# Autodesk Inventor assembly: Box_assembly
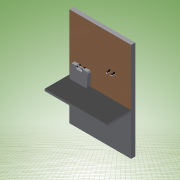
[picture p0: Inventor's stored thumbnail of the model, 180x180]
Saved by Autodesk Inventor 2017 (Build 210142000, 142)
## iProperties
Created: 2018-06-04
Part Number: Box_assembly
Document SubType Name: Assembly
Designer: Spark Electronics
Author: Spark Electronics
## Documents named in this file (5)
- C:\Users\Owner\Documents\SPARK RESEARCH\Projects\Organization\Divider Boxes\Box_assembly.iam
- C:\Users\Owner\Documents\SPARK RESEARCH\Projects\Organization\Divider Boxes\Wall_desk.ipt
- C:\Users\Owner\Documents\SPARK RESEARCH\Projects\Organization\Divider Boxes\Divider_box.ipt
- C:\Users\Owner\Documents\SPARK RESEARCH\Projects\Organization\Divider Boxes\wall_hook.ipt
- C:\Users\Owner\Documents\SPARK RESEARCH\Projects\Organization\Divider Boxes\Wall_mount.ipt
## Components (8 placed, 4 different names)
1. Wall_desk:1 — Mate:1, Mate:2, Flush:6, Mate:11, Mate:12
2. Divider_box:1 — Mate:5, Mate:7, Mate:8, Mate:9, Mate:10
3. wall_hook:1 — Flush:5, Mate:6, Mate:7, Mate:8, Mate:13, Mate:14, Mate:15
4. wall_hook:2 — Flush:5, Mate:5, Mate:6, Flush:6, Mate:9, Mate:10
5. wall_hook:3 — Mate:2
6. wall_hook:4 — Mate:1
7. Wall_mount:1 — Mate:12, Flush:7, Mate:13, Mate:14, Mate:15
8. Wall_mount:2 — Mate:11, Flush:7
## Relationships (16: Mate 13, Flush 3)
- Mate:1: Wall_desk:1 ↔ wall_hook:4
- Mate:2: Wall_desk:1 ↔ wall_hook:3
- Flush:5: wall_hook:1 ↔ wall_hook:2
- Mate:5: Divider_box:1 ↔ wall_hook:2
- Mate:6 (101.6 mm): wall_hook:1 ↔ wall_hook:2
- Mate:7 (0.254 mm): Divider_box:1 ↔ wall_hook:1
- Mate:8: Divider_box:1 ↔ wall_hook:1
- Flush:6 (381 mm): Wall_desk:1 ↔ wall_hook:2
- Mate:9 (6.35 mm): Divider_box:1 ↔ wall_hook:2
- Mate:10 (0.254 mm): Divider_box:1 ↔ wall_hook:2
- Mate:11: Wall_desk:1 ↔ Wall_mount:2
- Mate:12: Wall_desk:1 ↔ Wall_mount:1
- Flush:7 (6.35 mm): Wall_mount:1 ↔ Wall_mount:2
- Mate:13 (0.1 mm): wall_hook:1 ↔ Wall_mount:1
- Mate:14 (0.1 mm): wall_hook:1 ↔ Wall_mount:1
- Mate:15 (0.1 mm): wall_hook:1 ↔ Wall_mount:1
